# Autodesk Inventor assembly: HoloscopeRaspberry
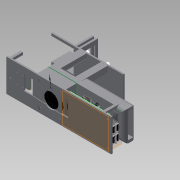
[picture p0: Inventor's stored thumbnail of the model, 180x180]
Saved by Autodesk Inventor 2015 (Build 190159000, 159)
## iProperties
Created: 2016-03-06
Part Number: HoloscopeRaspberry
Document SubType Name: Assembly
Designer: Bene
Author: Bene
## Documents named in this file (13)
- C:\Users\Bene\Dropbox\Dokumente\FHKoeln\Projekt_OE\Inventor\HoloscopeRaspberry\HoloscopeRaspberry.iam
- C:\Users\Bene\Dropbox\Dokumente\FHKoeln\Projekt_OE\Inventor\HoloscopeRaspberry\Importierte Komponenten\RaspberryPi2 STEP214\RaspberryPi2 STEP214.iam
- C:\Users\Bene\Dropbox\Dokumente\FHKoeln\Projekt_OE\Inventor\HoloscopeRaspberry\Importierte Komponenten\RasPi_Camera\RasPi_Camera.iam
- C:\Users\Bene\Dropbox\Dokumente\FHKoeln\Projekt_OE\Inventor\HoloscopeRaspberry\SonyQX_Mechanik.iam
- C:\Users\Bene\Dropbox\Dokumente\FHKoeln\Projekt_OE\Inventor\HoloscopeRaspberry\00_Anker.ipt
- C:\Users\Bene\Dropbox\Dokumente\FHKoeln\Projekt_OE\Inventor\HoloscopeRaspberry\10_Grundplatte.ipt
- C:\Users\Bene\Dropbox\Dokumente\FHKoeln\Projekt_OE\Inventor\HoloscopeRaspberry\11_Stange.ipt
- C:\Users\Bene\Dropbox\Dokumente\FHKoeln\Projekt_OE\Inventor\HoloscopeRaspberry\20_Schlitten.ipt
- C:\Users\Bene\Dropbox\Dokumente\FHKoeln\Projekt_OE\Inventor\HoloscopeRaspberry\12_Zwischenebene_Akku.ipt
- C:\Users\Bene\Dropbox\Dokumente\FHKoeln\Projekt_OE\Inventor\HoloscopeRaspberry\11_Objektaufnahme.ipt
- C:\Users\Bene\Dropbox\Dokumente\FHKoeln\Projekt_OE\Inventor\HoloscopeRaspberry\13_Zwischenebene_LCD.ipt
- C:\Users\Bene\Dropbox\Dokumente\FHKoeln\Projekt_OE\Inventor\HoloscopeRaspberry\07_Feder.ipt
- C:\Users\Bene\Dropbox\Dokumente\FHKoeln\Projekt_OE\Inventor\HoloscopeRaspberry\90_Linearführung.ipt
## Components (15 placed, 12 different names)
1. RaspberryPi2 STEP214:1 [sub-assembly] — Fluchtend:1, Fluchtend:2, Fluchtend:4
2. SonyQX_Mechanik:1 [sub-assembly] — Passend:1, Passend:2
3. 00_Anker:1 — Fluchtend:14
4. RasPi_Camera:3 [sub-assembly] — Passend:3, Fluchtend:4, Fluchtend:15, Passend:6
5. 10_Grundplatte:1 — Fluchtend:1, Fluchtend:2, Passend:1, Passend:2, Passend:3, Fluchtend:11, Fluchtend:12, Fluchtend:14, Fluchtend:15, Fluchtend:17, Passend:10
6. 11_Stange:1
7. 11_Stange:2
8. 11_Stange:3
9. 11_Stange:4
10. 20_Schlitten:1 — Passend:7, Fluchtend:16, Passend:8
11. 12_Zwischenebene_Akku:1 — Fluchtend:11, Fluchtend:12, Passend:11
12. 11_Objektaufnahme:1 — Passend:6, Passend:7, Fluchtend:16
13. 13_Zwischenebene_LCD:1 — Passend:11
14. 07_Feder:1 — Passend:8
15. 90_Linearführung:1 — Fluchtend:17, Passend:10
## Relationships (17: Flush 9, Mate 8)
- Fluchtend:1 [Flush]: RaspberryPi2 STEP214:1 ↔ 10_Grundplatte:1
- Fluchtend:2 [Flush] (8 mm): RaspberryPi2 STEP214:1 ↔ 10_Grundplatte:1
- Passend:1 [Mate]: SonyQX_Mechanik:1 ↔ 10_Grundplatte:1
- Passend:2 [Mate]: SonyQX_Mechanik:1 ↔ 10_Grundplatte:1
- Passend:3 [Mate] (1 mm): RasPi_Camera:3 ↔ 10_Grundplatte:1
- Fluchtend:4 [Flush] (-10 mm): RaspberryPi2 STEP214:1 ↔ RasPi_Camera:3
- Fluchtend:11 [Flush]: 10_Grundplatte:1 ↔ 12_Zwischenebene_Akku:1
- Fluchtend:12 [Flush]: 10_Grundplatte:1 ↔ 12_Zwischenebene_Akku:1
- Fluchtend:14 [Flush]: 00_Anker:1 ↔ 10_Grundplatte:1
- Fluchtend:15 [Flush]: RasPi_Camera:3 ↔ 10_Grundplatte:1
- Passend:6 [Mate] (1 mm): RasPi_Camera:3 ↔ 11_Objektaufnahme:1
- Passend:7 [Mate]: 20_Schlitten:1 ↔ 11_Objektaufnahme:1
- Fluchtend:16 [Flush]: 20_Schlitten:1 ↔ 11_Objektaufnahme:1
- Passend:8 [Mate]: 20_Schlitten:1 ↔ 07_Feder:1
- Fluchtend:17 [Flush] (2 mm): 10_Grundplatte:1 ↔ 90_Linearführung:1
- Passend:10 [Mate] (1 mm): 10_Grundplatte:1 ↔ 90_Linearführung:1
- Passend:11 [Mate]: 12_Zwischenebene_Akku:1 ↔ 13_Zwischenebene_LCD:1
